# Autodesk Inventor assembly: Assembly_Matchboxscope_injectionmolded
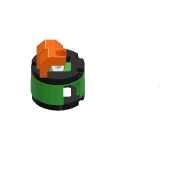
[picture p0: Inventor's stored thumbnail of the model, 180x180]
Saved by Autodesk Inventor 2022 (Build 260153000, 153)
## iProperties
Created: 2023-04-12
Part Number: Assembly_Matchboxscope_injectionmolded
Document SubType Name: Assembly
Designer: diederichbenedict
Author: diederichbenedict
## Documents named in this file (6)
- C:\Users\diederichbenedict\Dropbox\Dokumente\Promotion\PROJECTS\Matchboxscope\INVENTOR\RELEASE\Matchboxscope\Workspace\Assembly_Matchboxscope_injectionmolded.iam
- C:\Users\diederichbenedict\Dropbox\Dokumente\Promotion\PROJECTS\Matchboxscope\INVENTOR\RELEASE\Matchboxscope\Workspace\IM_Matchboxscope_base.ipt
- C:\Users\diederichbenedict\Dropbox\Dokumente\Promotion\PROJECTS\Matchboxscope\INVENTOR\RELEASE\Matchboxscope\Workspace\IM_Matchboxscope_plate.ipt
- C:\Users\diederichbenedict\Dropbox\Dokumente\Promotion\PROJECTS\Matchboxscope\INVENTOR\RELEASE\Matchboxscope\Workspace\IM_Lensholder.ipt
- C:\Users\diederichbenedict\Dropbox\Dokumente\Promotion\PROJECTS\Matchboxscope\INVENTOR\RELEASE\Matchboxscope\Workspace\IM_Periscope.ipt
- C:\Users\diederichbenedict\Dropbox\Dokumente\Promotion\PROJECTS\Matchboxscope\INVENTOR\RELEASE\Matchboxscope\Workspace\IM_ledholder.ipt
## Components (6 placed, 5 different names)
1. IM_Matchboxscope_base:1 — Fluchtend:1
2. IM_Matchboxscope_plate:1
3. IM_Matchboxscope_plate:2 — Einfügen:4, Winkel:1
4. IM_Lensholder:1 — Fluchtend:1
5. IM_Periscope:1 — Einfügen:4, Winkel:1
6. IM_ledholder:1
## Relationships (7: Insert 4, Mate 1, Flush 1, Angle 1)
- [Insert]: IM_Matchboxscope_base:1 ↔ IM_Matchboxscope_plate:1
- [Insert]: IM_Matchboxscope_base:1 ↔ IM_Matchboxscope_plate:1
- [Insert]: IM_Matchboxscope_base:1 ↔ IM_Matchboxscope_plate:2
- [Mate]: IM_Matchboxscope_base:1 ↔ IM_Matchboxscope_plate:2
- Fluchtend:1 [Flush]: IM_Matchboxscope_base:1 ↔ IM_Lensholder:1
- Einfügen:4 [Insert]: IM_Matchboxscope_plate:2 ↔ IM_Periscope:1
- Winkel:1 [Angle] (0 deg): IM_Matchboxscope_plate:2 ↔ IM_Periscope:1
